# Autodesk Inventor assembly: 꼽게+센서(최종으로가는과정)
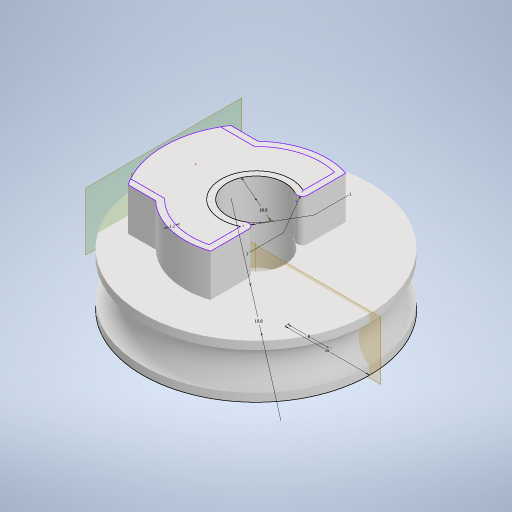
[picture p0: Inventor's stored thumbnail of the model, 512x512]
Saved by Autodesk Inventor 2023 (Build 270158000, 158)
## iProperties
Created: 2023-04-25
Part Number: 꼽게+센서(최종으로가는과정)
Document SubType Name: Assembly
Designer: rlatk
Author: rlatk
## Documents named in this file (3)
- C:\Users\rlatk\Desktop\코일건\코일건 부품\꼽게+센서(최종으로가는과정).iam
- C:\Users\rlatk\Desktop\코일건\코일건 부품\ir다이오드4.ipt
- C:\Users\rlatk\Desktop\코일건\코일건 부품\코일건원통꼽게1.ipt
## Components (2 placed, 2 different names)
1. ir다이오드4:1 — 회전:1
2. 코일건원통꼽게1:1 — 회전:1
## Relationships (1: RevoluteJoint 1)
- 회전:1 [RevoluteJoint]: ir다이오드4:1 ↔ 코일건원통꼽게1:1
